# Autodesk Inventor assembly: Assembly_Opentrons_Imagingunit_v3
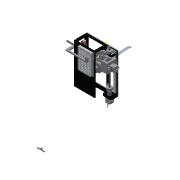
[picture p0: Inventor's stored thumbnail of the model, 180x180]
Saved by Autodesk Inventor 2019.4 (Build 234330000, 330)
## iProperties
Created: 2021-01-31
Part Number: Assembly_Opentrons_Imagingunit_v3
Document SubType Name: Assembly
Designer: diederichbenedict
Author: diederichbenedict
## Documents named in this file (7)
- C:\Users\diederichbenedict\Dropbox\Dokumente\Promotion\PROJECTS\OPENTRONS\INVENTOR\Assembly_Opentrons_Imagingunit_v3.iam
- C:\Users\diederichbenedict\Dropbox\Dokumente\Promotion\PROJECTS\OPENTRONS\INVENTOR\Assembly_opentrons_microscope_slide_y_base.iam
- C:\Users\diederichbenedict\Dropbox\Dokumente\Promotion\PROJECTS\OPENTRONS\INVENTOR\Assembly_opentrons_microscope_slide_y.iam
- C:\Users\diederichbenedict\Dropbox\Dokumente\Promotion\PROJECTS\OPENTRONS\INVENTOR\Assembly_Opentrons_Autofocus_v2.iam
- C:\Users\diederichbenedict\Dropbox\Dokumente\Promotion\PROJECTS\OPENTRONS\INVENTOR\00_MTP_96-welplate.ipt
- C:\Users\diederichbenedict\Dropbox\Dokumente\Promotion\PROJECTS\OPENTRONS\INVENTOR\04_OPENTRONS_Microscope_wellplate_base.ipt
- C:\Users\diederichbenedict\Dropbox\Dokumente\Promotion\PROJECTS\OPENTRONS\INVENTOR\06_Fluorescence_Arm.ipt
## Components (6 placed, 6 different names)
1. Assembly_opentrons_microscope_slide_y_base:1 [sub-assembly] — Mate:10, Mate:11, Mate:12, Angle:6, Angle:7
2. Assembly_Opentrons_Autofocus_v2:1 [sub-assembly] — Mate:13, Flush:1, Flush:2
3. 00_MTP_96-welplate:1 — Mate:10, Mate:11, Mate:14
4. Assembly_opentrons_microscope_slide_y:1 [sub-assembly] — Mate:12, Angle:6, Mate:13, Angle:7
5. 04_OPENTRONS_Microscope_wellplate_base:1 — Mate:14
6. 06_Fluorescence_Arm:1 — Flush:1, Flush:2
## Relationships (11: Mate 5, Angle 4, Flush 2)
- [Angle] (180 deg): Assembly_opentrons_microscope_slide_y_base:1 ↔ Assembly_Opentrons_Autofocus_v2:1
- Mate:10: Assembly_opentrons_microscope_slide_y_base:1 ↔ 00_MTP_96-welplate:1
- Mate:11 (10 mm): Assembly_opentrons_microscope_slide_y_base:1 ↔ 00_MTP_96-welplate:1
- [Angle] (180 deg): Assembly_opentrons_microscope_slide_y_base:1 ↔ Assembly_Opentrons_Autofocus_v2:1
- Mate:12: Assembly_opentrons_microscope_slide_y_base:1 ↔ Assembly_opentrons_microscope_slide_y:1
- Angle:6 (180 deg): Assembly_opentrons_microscope_slide_y_base:1 ↔ Assembly_opentrons_microscope_slide_y:1
- Mate:13: Assembly_Opentrons_Autofocus_v2:1 ↔ Assembly_opentrons_microscope_slide_y:1
- Angle:7 (180 deg): Assembly_opentrons_microscope_slide_y_base:1 ↔ Assembly_opentrons_microscope_slide_y:1
- Mate:14: 00_MTP_96-welplate:1 ↔ 04_OPENTRONS_Microscope_wellplate_base:1
- Flush:1: Assembly_Opentrons_Autofocus_v2:1 ↔ 06_Fluorescence_Arm:1
- Flush:2: Assembly_Opentrons_Autofocus_v2:1 ↔ 06_Fluorescence_Arm:1
